# Autodesk Inventor assembly: caixa
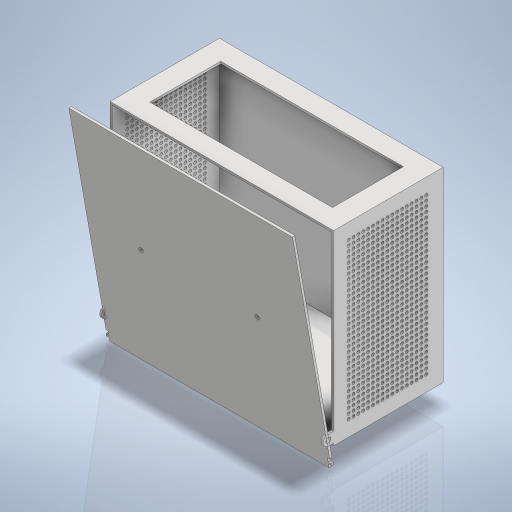
[picture p0: Inventor's stored thumbnail of the model, 512x512]
Saved by Autodesk Inventor 2024.3 (Build 283343000, 343)
## iProperties
Created: 2024-04-25
Part Number: caixa
Document SubType Name: Assembly
Designer: joaov
Author: joaov
## Documents named in this file (3)
- D:\Downloads\artigo\modelo_caixa\caixa.iam
- D:\Downloads\dry_box\caixa.ipt
- D:\Downloads\artigo\modelo_caixa\tampa.ipt
## Components (2 placed, 2 different names)
1. caixa:1 — Ângulo:1, Coincidente:1
2. tampa:1 — Ângulo:1, Coincidente:1
## Relationships (2: Angle 1, Mate 1)
- Ângulo:1 [Angle] (10 deg): caixa:1 ↔ tampa:1
- Coincidente:1 [Mate]: caixa:1 ↔ tampa:1
